# Autodesk Inventor assembly: ASY DS-B beam 3
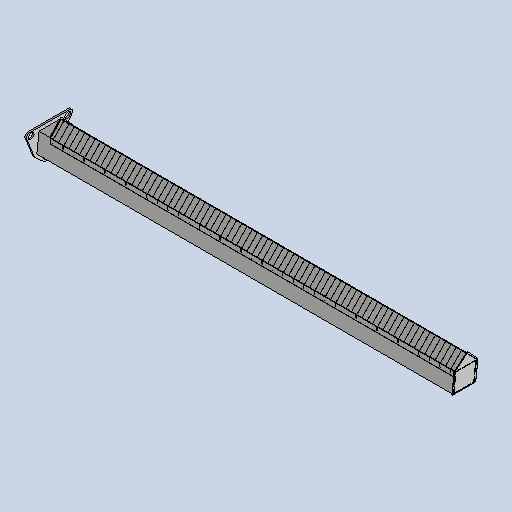
[picture p0: Inventor's stored thumbnail of the model, 512x512]
Saved by Autodesk Inventor 2025.1 (Build 291241020, 241B)
## iProperties
Created: 2025-02-18
Part Number: ASY DS-B beam 3
Document SubType Name: Assembly
Designer: admin
Author: admin
## Documents named in this file (6)
- C:\Users\user\YandexDisk-badmisterfox\home pc\Inventor\Manturovo\Manturovo_Se-clar\Дренаж на угольные\2200\ASY DS-B beam 3.iam
- C:\Users\user\YandexDisk-badmisterfox\home pc\Inventor\Manturovo\Manturovo_Se-clar\Дренаж на угольные\2200\DSB-503 beam 3.ipt
- C:\Users\user\YandexDisk-badmisterfox\home pc\Inventor\Manturovo\Manturovo_Se-clar\Дренаж на угольные\2200\DSB-513 roof 3.ipt
- C:\Users\user\YandexDisk-badmisterfox\home pc\Inventor\Manturovo\Manturovo_Se-clar\Дренаж на угольные\2200\DSB-507 beam flange.ipt
- C:\Users\user\YandexDisk-badmisterfox\home pc\Inventor\Manturovo\Manturovo_Se-clar\Дренаж на угольные\2200\DSB-508 CAP house.ipt
- C:\Users\user\YandexDisk-badmisterfox\home pc\Inventor\Manturovo\Manturovo_Se-clar\Дренаж на угольные\2200\DSB-509 CAP roof.ipt
## Components (5 placed, 5 different names)
1. DSB-503 beam 3:1 — Mate:2, Flush:3, Flush:4, Flush:1, Mate:1, Flush:6, Mate:6, Rigid:1, Rigid:2
2. DSB-513 roof 3:1 — Flush:1, Mate:1, Flush:6, Mate:7
3. DSB-507 beam flange:1 — Rigid:1
4. DSB-508 CAP house:1 — Mate:3, Rigid:2
5. DSB-509 CAP roof:1 — Mate:5, Mate:6, Mate:7
## Relationships (12: Mate 6, Flush 4, WeldJoint 2)
- Mate:2: DSB-503 beam 3:1
- Flush:3: DSB-503 beam 3:1
- Flush:4: DSB-503 beam 3:1
- Flush:1: DSB-503 beam 3:1 ↔ DSB-513 roof 3:1
- Mate:1: DSB-503 beam 3:1 ↔ DSB-513 roof 3:1
- Flush:6: DSB-503 beam 3:1 ↔ DSB-513 roof 3:1
- Mate:3: DSB-508 CAP house:1
- Mate:5: DSB-509 CAP roof:1
- Mate:6: DSB-503 beam 3:1 ↔ DSB-509 CAP roof:1
- Mate:7: DSB-513 roof 3:1 ↔ DSB-509 CAP roof:1
- Rigid:1 [WeldJoint]: DSB-503 beam 3:1 ↔ DSB-507 beam flange:1
- Rigid:2 [WeldJoint]: DSB-503 beam 3:1 ↔ DSB-508 CAP house:1
